# Autodesk Inventor assembly: Chasis Montaje
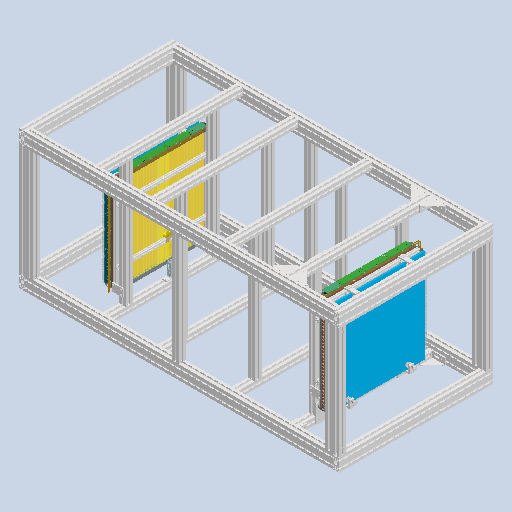
[picture p0: Inventor's stored thumbnail of the model, 512x512]
Saved by Autodesk Inventor 2024.2 (Build 282272000, 272)
## iProperties
Created: 2025-06-05
Part Number: Chasis Montaje
Document SubType Name: Assembly
Designer: ja.restrepo1
Author: ja.restrepo1
## Documents named in this file (9)
- I:\MICROMECANICA\ALTAS ENERGIAS\Deteccion de Muones\Detectores centelladores\Partes Detectores centelladores\Chasis DC\Chasis Montaje.iam
- I:\MICROMECANICA\ALTAS ENERGIAS\Deteccion de Muones\Detectores centelladores\Partes Detectores centelladores\Chasis DC\SE. Chasis DC.iam
- I:\MICROMECANICA\ALTAS ENERGIAS\Deteccion de Muones\Detectores centelladores\Partes Detectores centelladores\PARTES DC\EG Detector Centellador.iam
- I:\MICROMECANICA\ALTAS ENERGIAS\Deteccion de Muones\Detectores centelladores\Partes Detectores centelladores\Chasis DC\Partes Chasis DC\Soporte.ipt
- I:\MICROMECANICA\ALTAS ENERGIAS\Deteccion de Muones\Detectores centelladores\Partes Detectores centelladores\Chasis DC\Partes Chasis DC\Lamina centelladora.ipt
- I:\MICROMECANICA\ALTAS ENERGIAS\Deteccion de Muones\Detectores centelladores\Partes Detectores centelladores\Chasis DC\Partes Chasis DC\Sujecion centelladora.iam
- I:\MICROMECANICA\ALTAS ENERGIAS\Deteccion de Muones\Detectores centelladores\Partes Detectores centelladores\PARTES DC\Tarjetas IC DC\SE tarjedas de AD DC.iam
- I:\MICROMECANICA\ALTAS ENERGIAS\Deteccion de Muones\Detectores centelladores\Partes Detectores centelladores\PARTES DC\Tarjetas IC DC\unión placa soporte TIC DC.ipt
- I:\MICROMECANICA\ALTAS ENERGIAS\Deteccion de Muones\Detectores centelladores\Partes Detectores centelladores\Chasis DC\Partes Chasis DC\SE. fuente.iam
## Components (27 placed, 8 different names)
1. SE. Chasis DC:1 [sub-assembly] — Nivelación:1, Nivelación:2, Nivelación:3, Coincidencia:1, Ángulo:1, Ángulo:2, Coincidencia:5, Coincidencia:6, Coincidencia:7, Nivelación:7, Coincidencia:10, Coincidencia:12, Coincidencia:14, Coincidencia:16, Coincidencia:24, Coincidencia:25, Coincidencia:26, Coincidencia:27, Coincidencia:28, Coincidencia:29, Coincidencia:30, Coincidencia:31, Coincidencia:74, Nivelación:25, Coincidencia:75, Nivelación:26
2. EG Detector Centellador:1 [sub-assembly] — Ángulo:1, Coincidencia:5, Nivelación:5, Nivelación:6, Coincidencia:6, Coincidencia:40, Nivelación:22, Coincidencia:41, Coincidencia:61, Nivelación:24, Coincidencia:62, Coincidencia:63, Coincidencia:65, Coincidencia:66, Coincidencia:67, Coincidencia:68, Coincidencia:69, Coincidencia:70, Coincidencia:71, Coincidencia:72, Coincidencia:73, Coincidencia:76, Coincidencia:77
3. EG Detector Centellador:2 [sub-assembly] — Ángulo:2, Nivelación:5, Nivelación:6, Coincidencia:7, Nivelación:7, Coincidencia:8, Coincidencia:9, Coincidencia:11, Nivelación:8, Coincidencia:13, Coincidencia:15, Coincidencia:23, Nivelación:16, Nivelación:17, Coincidencia:42, Coincidencia:43, Coincidencia:44, Coincidencia:45, Coincidencia:46, Coincidencia:47, Coincidencia:48, Coincidencia:49, Coincidencia:50, Coincidencia:51, Coincidencia:52, Coincidencia:53, Coincidencia:54, Nivelación:23
4. Soporte:1 — Coincidencia:8, Coincidencia:9, Coincidencia:12, Nivelación:10
5. Soporte:2 — Coincidencia:10, Coincidencia:11, Nivelación:8, Nivelación:9, Nivelación:13
6. Soporte:3 — Coincidencia:13, Coincidencia:14, Nivelación:9, Nivelación:15
7. Soporte:4 — Coincidencia:15, Coincidencia:16, Nivelación:10, Nivelación:14
8. Lamina centelladora:1 — Coincidencia:23, Nivelación:16, Nivelación:17
9. Soporte:5 — Coincidencia:26, Coincidencia:27, Nivelación:13
10. Soporte:6 — Coincidencia:24, Coincidencia:25, Coincidencia:76
11. Soporte:7 — Coincidencia:28, Coincidencia:29, Nivelación:14
12. Soporte:8 — Coincidencia:30, Coincidencia:31, Nivelación:15
13. Lamina centelladora:2 — Coincidencia:40, Nivelación:22, Coincidencia:41
14. Sujecion centelladora:1 [sub-assembly] — Coincidencia:42, Coincidencia:43, Coincidencia:44
15. Sujecion centelladora:2 [sub-assembly] — Coincidencia:48, Coincidencia:49, Coincidencia:50
16. Sujecion centelladora:4 [sub-assembly] — Coincidencia:45, Coincidencia:46, Coincidencia:47
17. Sujecion centelladora:6 [sub-assembly] — Coincidencia:51, Coincidencia:52, Coincidencia:53
18. SE tarjedas de AD DC:1 [sub-assembly] — Coincidencia:55, Coincidencia:56, Coincidencia:57
19. unión placa soporte TIC DC:1 — Coincidencia:54, Nivelación:23, Coincidencia:55, Coincidencia:56, Coincidencia:57
20. SE tarjedas de AD DC:2 [sub-assembly]
21. unión placa soporte TIC DC:2 — Coincidencia:61, Nivelación:24
22. Sujecion centelladora:7 [sub-assembly] — Coincidencia:62, Coincidencia:63, Coincidencia:77
23. Sujecion centelladora:8 [sub-assembly] — Coincidencia:65, Coincidencia:66, Coincidencia:67
24. Sujecion centelladora:9 [sub-assembly] — Coincidencia:68, Coincidencia:69, Coincidencia:70
25. Sujecion centelladora:10 [sub-assembly] — Coincidencia:71, Coincidencia:72, Coincidencia:73
26. SE. fuente:1 [sub-assembly] — Coincidencia:74, Nivelación:25
27. SE. fuente:2 [sub-assembly] — Coincidencia:75, Nivelación:26
## Relationships (80: Mate 59, Flush 19, Angle 2)
- Nivelación:1 [Flush]: SE. Chasis DC:1
- Nivelación:2 [Flush]: SE. Chasis DC:1
- Nivelación:3 [Flush]: SE. Chasis DC:1
- Coincidencia:1 [Mate]: SE. Chasis DC:1
- Ángulo:1 [Angle] (0 deg): SE. Chasis DC:1 ↔ EG Detector Centellador:1
- Ángulo:2 [Angle] (0 deg): SE. Chasis DC:1 ↔ EG Detector Centellador:2
- Coincidencia:5 [Mate] (10 mm): SE. Chasis DC:1 ↔ EG Detector Centellador:1
- Nivelación:5 [Flush]: EG Detector Centellador:1 ↔ EG Detector Centellador:2
- Nivelación:6 [Flush]: EG Detector Centellador:1 ↔ EG Detector Centellador:2
- Coincidencia:6 [Mate]: SE. Chasis DC:1 ↔ EG Detector Centellador:1
- Coincidencia:7 [Mate]: SE. Chasis DC:1 ↔ EG Detector Centellador:2
- Nivelación:7 [Flush]: SE. Chasis DC:1 ↔ EG Detector Centellador:2
- Coincidencia:8 [Mate]: EG Detector Centellador:2 ↔ Soporte:1
- Coincidencia:9 [Mate]: EG Detector Centellador:2 ↔ Soporte:1
- Coincidencia:10 [Mate]: SE. Chasis DC:1 ↔ Soporte:2
- Coincidencia:11 [Mate]: EG Detector Centellador:2 ↔ Soporte:2
- Coincidencia:12 [Mate] (50 mm): SE. Chasis DC:1 ↔ Soporte:1
- Nivelación:8 [Flush] (50 mm): EG Detector Centellador:2 ↔ Soporte:2
- Coincidencia:13 [Mate]: EG Detector Centellador:2 ↔ Soporte:3
- Coincidencia:14 [Mate]: SE. Chasis DC:1 ↔ Soporte:3
- Nivelación:9 [Flush]: Soporte:2 ↔ Soporte:3
- Coincidencia:15 [Mate]: EG Detector Centellador:2 ↔ Soporte:4
- Coincidencia:16 [Mate]: SE. Chasis DC:1 ↔ Soporte:4
- Nivelación:10 [Flush]: Soporte:1 ↔ Soporte:4
- Coincidencia:23 [Mate]: EG Detector Centellador:2 ↔ Lamina centelladora:1
- Coincidencia:24 [Mate]: SE. Chasis DC:1 ↔ Soporte:6
- Coincidencia:25 [Mate]: SE. Chasis DC:1 ↔ Soporte:6
- Coincidencia:26 [Mate]: SE. Chasis DC:1 ↔ Soporte:5
- Coincidencia:27 [Mate]: SE. Chasis DC:1 ↔ Soporte:5
- Nivelación:13 [Flush]: Soporte:2 ↔ Soporte:5
- Coincidencia:28 [Mate]: SE. Chasis DC:1 ↔ Soporte:7
- Coincidencia:29 [Mate]: SE. Chasis DC:1 ↔ Soporte:7
- Nivelación:14 [Flush]: Soporte:4 ↔ Soporte:7
- Coincidencia:30 [Mate]: SE. Chasis DC:1 ↔ Soporte:8
- Coincidencia:31 [Mate]: SE. Chasis DC:1 ↔ Soporte:8
- Nivelación:15 [Flush]: Soporte:3 ↔ Soporte:8
- Nivelación:16 [Flush]: EG Detector Centellador:2 ↔ Lamina centelladora:1
- Nivelación:17 [Flush]: EG Detector Centellador:2 ↔ Lamina centelladora:1
- Coincidencia:40 [Mate]: EG Detector Centellador:1 ↔ Lamina centelladora:2
- Nivelación:22 [Flush]: EG Detector Centellador:1 ↔ Lamina centelladora:2
- Coincidencia:41 [Mate]: EG Detector Centellador:1 ↔ Lamina centelladora:2
- Coincidencia:42 [Mate]: EG Detector Centellador:2 ↔ Sujecion centelladora:1
- Coincidencia:43 [Mate]: EG Detector Centellador:2 ↔ Sujecion centelladora:1
- Coincidencia:44 [Mate]: EG Detector Centellador:2 ↔ Sujecion centelladora:1
- Coincidencia:45 [Mate]: EG Detector Centellador:2 ↔ Sujecion centelladora:4
- Coincidencia:46 [Mate]: EG Detector Centellador:2 ↔ Sujecion centelladora:4
- Coincidencia:47 [Mate]: EG Detector Centellador:2 ↔ Sujecion centelladora:4
- Coincidencia:48 [Mate]: EG Detector Centellador:2 ↔ Sujecion centelladora:2
- Coincidencia:49 [Mate]: EG Detector Centellador:2 ↔ Sujecion centelladora:2
- Coincidencia:50 [Mate]: EG Detector Centellador:2 ↔ Sujecion centelladora:2
- Coincidencia:51 [Mate]: EG Detector Centellador:2 ↔ Sujecion centelladora:6
- Coincidencia:52 [Mate]: EG Detector Centellador:2 ↔ Sujecion centelladora:6
- Coincidencia:53 [Mate]: EG Detector Centellador:2 ↔ Sujecion centelladora:6
- Coincidencia:54 [Mate]: EG Detector Centellador:2 ↔ unión placa soporte TIC DC:1
- Nivelación:23 [Flush]: EG Detector Centellador:2 ↔ unión placa soporte TIC DC:1
- Coincidencia:55 [Mate]: SE tarjedas de AD DC:1 ↔ unión placa soporte TIC DC:1
- Coincidencia:56 [Mate]: SE tarjedas de AD DC:1 ↔ unión placa soporte TIC DC:1
- Coincidencia:57 [Mate]: SE tarjedas de AD DC:1 ↔ unión placa soporte TIC DC:1
- [Mate]: SE tarjedas de AD DC:2 ↔ unión placa soporte TIC DC:2
- [Mate]: SE tarjedas de AD DC:2 ↔ unión placa soporte TIC DC:2
- [Mate]: SE tarjedas de AD DC:2 ↔ unión placa soporte TIC DC:2
- Coincidencia:61 [Mate]: EG Detector Centellador:1 ↔ unión placa soporte TIC DC:2
- Nivelación:24 [Flush]: EG Detector Centellador:1 ↔ unión placa soporte TIC DC:2
- Coincidencia:62 [Mate]: EG Detector Centellador:1 ↔ Sujecion centelladora:7
- Coincidencia:63 [Mate]: EG Detector Centellador:1 ↔ Sujecion centelladora:7
- Coincidencia:65 [Mate]: EG Detector Centellador:1 ↔ Sujecion centelladora:8
- Coincidencia:66 [Mate]: EG Detector Centellador:1 ↔ Sujecion centelladora:8
- Coincidencia:67 [Mate]: EG Detector Centellador:1 ↔ Sujecion centelladora:8
- Coincidencia:68 [Mate]: EG Detector Centellador:1 ↔ Sujecion centelladora:9
- Coincidencia:69 [Mate]: EG Detector Centellador:1 ↔ Sujecion centelladora:9
- Coincidencia:70 [Mate]: EG Detector Centellador:1 ↔ Sujecion centelladora:9
- Coincidencia:71 [Mate]: EG Detector Centellador:1 ↔ Sujecion centelladora:10
- Coincidencia:72 [Mate]: EG Detector Centellador:1 ↔ Sujecion centelladora:10
- Coincidencia:73 [Mate]: EG Detector Centellador:1 ↔ Sujecion centelladora:10
- Coincidencia:74 [Mate]: SE. Chasis DC:1 ↔ SE. fuente:1
- Nivelación:25 [Flush] (7.5 mm): SE. Chasis DC:1 ↔ SE. fuente:1
- Coincidencia:75 [Mate]: SE. Chasis DC:1 ↔ SE. fuente:2
- Nivelación:26 [Flush] (7.5 mm): SE. Chasis DC:1 ↔ SE. fuente:2
- Coincidencia:76 [Mate] (50 mm): EG Detector Centellador:1 ↔ Soporte:6
- Coincidencia:77 [Mate]: EG Detector Centellador:1 ↔ Sujecion centelladora:7
## Named parameters: d124_d122 = 0 mm, d125_d123 = 0 mm, d126_d121 = 0 mm
